# Autodesk Inventor assembly: arduino uno
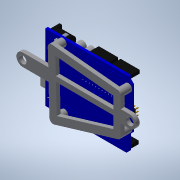
[picture p0: Inventor's stored thumbnail of the model, 180x180]
Saved by Autodesk Inventor 2020 (Build 240168000, 168)
## iProperties
Created: 2012-01-09
Part Number: arduino uno
Document SubType Name: Assembly
Designer: Trevor
Translation Standard: STEP AP214IS
FileName: Final.STEP
PreProcessor: SolidWorks 2011
PostProcessor: Build: 239, Release: 2011 RTM - Date: Wed 02/17/2010
Sent Units: millimeter
Uncertainty: 1e-05
Author: Trevor
## Documents named in this file (15)
- C:\Users\psrob\Desktop\arduino-uno.snapshot.3\arduino uno.iam
- C:\Users\psrob\Desktop\arduino-uno.snapshot.3\Stackable Female Pin Header_Default.ipt
- C:\Users\psrob\Desktop\arduino-uno.snapshot.3\Stackable Female Pin Header_6 Way.ipt
- C:\Users\psrob\Desktop\arduino-uno.snapshot.3\User Library-SOIC-8_Default.iam
- C:\Users\psrob\Desktop\arduino-uno.snapshot.3\User Library-ALU-D8_Default.iam
- C:\Users\psrob\Desktop\arduino-uno.snapshot.3\LED 1206_Default.ipt
- C:\Users\psrob\Desktop\arduino-uno.snapshot.3\Header Vertical 2.54mm Pitch2_Header 6 Way.ipt
- C:\Users\psrob\Desktop\arduino-uno.snapshot.3\SO 369A_Standard.ipt
- C:\Users\psrob\Desktop\arduino-uno.snapshot.3\XTAL Small_Default.ipt
- C:\Users\psrob\Desktop\arduino-uno.snapshot.3\User Library-QFN32 (FTDI)_Default.iam
- C:\Users\psrob\Desktop\arduino-uno.snapshot.3\User Library-dc range - dc connector[4840_2201]_Default.ipt
- C:\Users\psrob\Desktop\arduino-uno.snapshot.3\PCB_Final_Default.ipt
- C:\Users\psrob\Desktop\arduino-uno.snapshot.3\User Library-67068-0000-molex_Default.ipt
- C:\Users\psrob\Desktop\arduino-uno.snapshot.3\IC DIP 28_Default.ipt
- C:\Users\psrob\Desktop\arduino-uno.snapshot.3\uno_holder.ipt
## Components (20 placed, 14 different names)
1. Stackable Female Pin Header_Default:1
2. Stackable Female Pin Header_6 Way:1
3. User Library-SOIC-8_Default:1 [sub-assembly]
4. User Library-ALU-D8_Default:1 [sub-assembly]
5. User Library-ALU-D8_Default:2 [sub-assembly]
6. Stackable Female Pin Header_Default:2
7. LED 1206_Default:1
8. LED 1206_Default:2
9. Header Vertical 2.54mm Pitch2_Header 6 Way:1
10. SO 369A_Standard:1
11. Stackable Female Pin Header_6 Way:2
12. XTAL Small_Default:1
13. LED 1206_Default:3
14. User Library-QFN32 (FTDI)_Default:1 [sub-assembly]
15. User Library-dc range - dc connector[4840_2201]_Default:1
16. PCB_Final_Default:1 — Flush:1
17. LED 1206_Default:4
18. User Library-67068-0000-molex_Default:1
19. IC DIP 28_Default:1
20. uno_holder:1 — Flush:1
## Relationships (1: Flush 1)
- Flush:1: PCB_Final_Default:1 ↔ uno_holder:1
